# Autodesk Inventor assembly: ExtruderSatoer
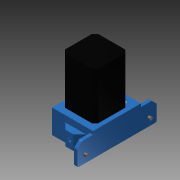
[picture p0: Inventor's stored thumbnail of the model, 180x180]
Saved by Autodesk Inventor 2015 SP1 (Build 190203100, 203)
## iProperties
Created: 2015-05-03
Part Number: ExtruderSatoer
Document SubType Name: Assembly
Designer: Jack
Author: Jack
## Documents named in this file (13)
- C:\Users\Jack\ownCloud\Projects\CrossBot\InventorModel\Extruder\ExtruderSatoer\ExtruderSatoerRight\ExtruderSatoerRight.iam
- C:\Users\Jack\ownCloud\Projects\CrossBot\InventorModel\Extruder\ExtruderSatoer\ExtruderSatoerRight\ExtruderSatoerBodyRight.ipt
- C:\Users\Jack\ownCloud\Projects\CrossBot\InventorModel\Extruder\ExtruderSatoer\ExtruderSatoerRight\ExtruderSatoerMotorMountRight.ipt
- C:\Users\Jack\ownCloud\Projects\CrossBot\InventorModel\Hardware\Bolts\SHCS\SHCS4\SHCS4x30.ipt
- C:\Users\Jack\ownCloud\Projects\CrossBot\InventorModel\Extruder\ExtruderSatoer\ExtruderSatoerRight\ExtruderSatoerBearingArmRight.ipt
- C:\Users\Jack\ownCloud\Projects\CrossBot\InventorModel\Extruder\ExtruderSatoer\ExtruderSatoerRight\ExtruderSatoerCamRight.ipt
- C:\Users\Jack\ownCloud\Projects\CrossBot\InventorModel\Extruder\ExtruderSatoer\ExtruderSatoerRight\ExtruderSatoerCamArmRight.ipt
- C:\Users\Jack\ownCloud\Projects\CrossBot\InventorModel\Hardware\Bearing\BearingRadialBall\BearingRadialBall624zz.ipt
- C:\Users\Jack\ownCloud\Projects\CrossBot\InventorModel\Hardware\Bolts\SHCS\SHCS4\SHCS4x12.ipt
- C:\Users\Jack\ownCloud\Projects\CrossBot\InventorModel\Hardware\Nuts\Nut4.ipt
- C:\Users\Jack\ownCloud\Projects\CrossBot\InventorModel\Hardware\BoltWashers\BoltWasher4\BoltWasher4x8.iam
- C:\Users\Jack\ownCloud\Projects\CrossBot\InventorModel\Hardware\Bolts\SHCS\SHCS3\SHCS3x12.ipt
- C:\Users\Jack\ownCloud\Projects\CrossBot\InventorModel\Electronics\Motors\StepperMotorNema17x60mm.ipt
## Components (21 placed, 12 different names)
1. ExtruderSatoerBodyRight:1 — Mate:4, Mate:5, Mate:6, Mate:7, Mate:8, Mate:9, Mate:13, Mate:15, Mate:16, Mate:22, Mate:23, Mate:24, Mate:25
2. ExtruderSatoerMotorMountRight:1 — Mate:29, Mate:30, Mate:31, Angle:2, Angle:3, Angle:4, Mate:32, Mate:33, Mate:34, Mate:35, Mate:36, Mate:37, Mate:38, Mate:39, Mate:40, Mate:42
3. ExtruderSatoerBearingArmRight:1 — Mate:10, Mate:11, Mate:12, Mate:13, Mate:18, Mate:19, Angle:1, Mate:21
4. ExtruderSatoerCamRight:1 — Mate:16, Mate:17
5. ExtruderSatoerCamArmRight:1 — Mate:14, Mate:15
6. BearingRadialBall624zz:1 — Mate:10, Mate:11
7. StepperMotorNema17x60mm:1 — Mate:40, Mate:41, Mate:42
8. SHCS3x12:4 — Mate:32, Mate:38, Mate:41
9. SHCS3x12:3 — Mate:35, Mate:36
10. SHCS3x12:2 — Mate:33, Mate:39
11. SHCS3x12:1 — Mate:34, Mate:37
12. Nut4:4 — Mate:28, Mate:29, Angle:4
13. Nut4:3 — Mate:27, Mate:30, Angle:3
14. Nut4:2 — Mate:26, Mate:31, Angle:2
15. BoltWasher4x8:2 [sub-assembly] — Mate:23, Mate:24
16. BoltWasher4x8:1 [sub-assembly] — Mate:22, Mate:25
17. Nut4:1 — Mate:20, Angle:1, Mate:21
18. SHCS4x12:1 — Mate:18, Mate:19, Mate:20
19. SHCS4x30:3 — Mate:4, Mate:9, Mate:17, Mate:27
20. SHCS4x30:2 — Mate:5, Mate:7, Mate:12, Mate:26
21. SHCS4x30:1 — Mate:6, Mate:8, Mate:14, Mate:28
## Relationships (46: Mate 42, Angle 4)
- [Mate] (0.25 mm): ExtruderSatoerBodyRight:1 ↔ ExtruderSatoerMotorMountRight:1
- [Mate] (0.25 mm): ExtruderSatoerBodyRight:1 ↔ ExtruderSatoerMotorMountRight:1
- [Mate]: ExtruderSatoerBodyRight:1 ↔ ExtruderSatoerMotorMountRight:1
- Mate:4: ExtruderSatoerBodyRight:1 ↔ SHCS4x30:3
- Mate:5: ExtruderSatoerBodyRight:1 ↔ SHCS4x30:2
- Mate:6: ExtruderSatoerBodyRight:1 ↔ SHCS4x30:1
- Mate:7: ExtruderSatoerBodyRight:1 ↔ SHCS4x30:2
- Mate:8: ExtruderSatoerBodyRight:1 ↔ SHCS4x30:1
- Mate:9: ExtruderSatoerBodyRight:1 ↔ SHCS4x30:3
- Mate:10: ExtruderSatoerBearingArmRight:1 ↔ BearingRadialBall624zz:1
- Mate:11: ExtruderSatoerBearingArmRight:1 ↔ BearingRadialBall624zz:1
- Mate:12: ExtruderSatoerBearingArmRight:1 ↔ SHCS4x30:2
- Mate:13 (0.15 mm): ExtruderSatoerBodyRight:1 ↔ ExtruderSatoerBearingArmRight:1
- Mate:14: ExtruderSatoerCamArmRight:1 ↔ SHCS4x30:1
- Mate:15 (0.15 mm): ExtruderSatoerBodyRight:1 ↔ ExtruderSatoerCamArmRight:1
- Mate:16 (0.15 mm): ExtruderSatoerBodyRight:1 ↔ ExtruderSatoerCamRight:1
- Mate:17: ExtruderSatoerCamRight:1 ↔ SHCS4x30:3
- Mate:18: ExtruderSatoerBearingArmRight:1 ↔ SHCS4x12:1
- Mate:19: ExtruderSatoerBearingArmRight:1 ↔ SHCS4x12:1
- Mate:20: Nut4:1 ↔ SHCS4x12:1
- Angle:1 (0 deg): ExtruderSatoerBearingArmRight:1 ↔ Nut4:1
- Mate:21: ExtruderSatoerBearingArmRight:1 ↔ Nut4:1
- Mate:22: ExtruderSatoerBodyRight:1 ↔ BoltWasher4x8:1
- Mate:23: ExtruderSatoerBodyRight:1 ↔ BoltWasher4x8:2
- Mate:24: ExtruderSatoerBodyRight:1 ↔ BoltWasher4x8:2
- Mate:25: ExtruderSatoerBodyRight:1 ↔ BoltWasher4x8:1
- Mate:26: Nut4:2 ↔ SHCS4x30:2
- Mate:27: Nut4:3 ↔ SHCS4x30:3
- Mate:28: Nut4:4 ↔ SHCS4x30:1
- Mate:29: ExtruderSatoerMotorMountRight:1 ↔ Nut4:4
- Mate:30: ExtruderSatoerMotorMountRight:1 ↔ Nut4:3
- Mate:31: ExtruderSatoerMotorMountRight:1 ↔ Nut4:2
- Angle:2 (0 deg): ExtruderSatoerMotorMountRight:1 ↔ Nut4:2
- Angle:3 (0 deg): ExtruderSatoerMotorMountRight:1 ↔ Nut4:3
- Angle:4 (0 deg): ExtruderSatoerMotorMountRight:1 ↔ Nut4:4
- Mate:32: ExtruderSatoerMotorMountRight:1 ↔ SHCS3x12:4
- Mate:33: ExtruderSatoerMotorMountRight:1 ↔ SHCS3x12:2
- Mate:34: ExtruderSatoerMotorMountRight:1 ↔ SHCS3x12:1
- Mate:35: ExtruderSatoerMotorMountRight:1 ↔ SHCS3x12:3
- Mate:36: ExtruderSatoerMotorMountRight:1 ↔ SHCS3x12:3
- Mate:37: ExtruderSatoerMotorMountRight:1 ↔ SHCS3x12:1
- Mate:38: ExtruderSatoerMotorMountRight:1 ↔ SHCS3x12:4
- Mate:39: ExtruderSatoerMotorMountRight:1 ↔ SHCS3x12:2
- Mate:40: ExtruderSatoerMotorMountRight:1 ↔ StepperMotorNema17x60mm:1
- Mate:41: StepperMotorNema17x60mm:1 ↔ SHCS3x12:4
- Mate:42: ExtruderSatoerMotorMountRight:1 ↔ StepperMotorNema17x60mm:1
